# Autodesk Inventor assembly: DesignRootModel^PCB_ESP32-C3-MINI-1_V1(2)_PCB_ESP32-C3-MINI-1_V1
(part 2 of 3)
- C:\Users\micyg\Projects\virtual_pet\VirtualBlob\Mechanical\boards\MainBoard\MainBoard_0_4_0\VirtualBlob_MainBoard_0.4.0\VirtualBlob_MainBoard_0.4.0\uid__1-169^DesignRootModel_PCB_ESP32-C3-MINI-1_V1(2)_PCB_ESP32.ipt
- C:\Users\micyg\Projects\virtual_pet\VirtualBlob\Mechanical\boards\MainBoard\MainBoard_0_4_0\VirtualBlob_MainBoard_0.4.0\VirtualBlob_MainBoard_0.4.0\uid__1-170^DesignRootModel_PCB_ESP32-C3-MINI-1_V1(2)_PCB_ESP32.ipt
- C:\Users\micyg\Projects\virtual_pet\VirtualBlob\Mechanical\boards\MainBoard\MainBoard_0_4_0\VirtualBlob_MainBoard_0.4.0\VirtualBlob_MainBoard_0.4.0\uid__1-171^DesignRootModel_PCB_ESP32-C3-MINI-1_V1(2)_PCB_ESP32.ipt
- C:\Users\micyg\Projects\virtual_pet\VirtualBlob\Mechanical\boards\MainBoard\MainBoard_0_4_0\VirtualBlob_MainBoard_0.4.0\VirtualBlob_MainBoard_0.4.0\uid__1-172^DesignRootModel_PCB_ESP32-C3-MINI-1_V1(2)_PCB_ESP32.ipt
- C:\Users\micyg\Projects\virtual_pet\VirtualBlob\Mechanical\boards\MainBoard\MainBoard_0_4_0\VirtualBlob_MainBoard_0.4.0\VirtualBlob_MainBoard_0.4.0\uid__1-173^DesignRootModel_PCB_ESP32-C3-MINI-1_V1(2)_PCB_ESP32.ipt
- C:\Users\micyg\Projects\virtual_pet\VirtualBlob\Mechanical\boards\MainBoard\MainBoard_0_4_0\VirtualBlob_MainBoard_0.4.0\VirtualBlob_MainBoard_0.4.0\uid__1-174^DesignRootModel_PCB_ESP32-C3-MINI-1_V1(2)_PCB_ESP32.ipt
- C:\Users\micyg\Projects\virtual_pet\VirtualBlob\Mechanical\boards\MainBoard\MainBoard_0_4_0\VirtualBlob_MainBoard_0.4.0\VirtualBlob_MainBoard_0.4.0\uid__1-175^DesignRootModel_PCB_ESP32-C3-MINI-1_V1(2)_PCB_ESP32.ipt
- C:\Users\micyg\Projects\virtual_pet\VirtualBlob\Mechanical\boards\MainBoard\MainBoard_0_4_0\VirtualBlob_MainBoard_0.4.0\VirtualBlob_MainBoard_0.4.0\uid__1-176^DesignRootModel_PCB_ESP32-C3-MINI-1_V1(2)_PCB_ESP32.ipt
- C:\Users\micyg\Projects\virtual_pet\VirtualBlob\Mechanical\boards\MainBoard\MainBoard_0_4_0\VirtualBlob_MainBoard_0.4.0\VirtualBlob_MainBoard_0.4.0\uid__1-177^DesignRootModel_PCB_ESP32-C3-MINI-1_V1(2)_PCB_ESP32.ipt
- C:\Users\micyg\Projects\virtual_pet\VirtualBlob\Mechanical\boards\MainBoard\MainBoard_0_4_0\VirtualBlob_MainBoard_0.4.0\VirtualBlob_MainBoard_0.4.0\uid__1-178^DesignRootModel_PCB_ESP32-C3-MINI-1_V1(2)_PCB_ESP32.ipt
- C:\Users\micyg\Projects\virtual_pet\VirtualBlob\Mechanical\boards\MainBoard\MainBoard_0_4_0\VirtualBlob_MainBoard_0.4.0\VirtualBlob_MainBoard_0.4.0\uid__1-179^DesignRootModel_PCB_ESP32-C3-MINI-1_V1(2)_PCB_ESP32.ipt
- C:\Users\micyg\Projects\virtual_pet\VirtualBlob\Mechanical\boards\MainBoard\MainBoard_0_4_0\VirtualBlob_MainBoard_0.4.0\VirtualBlob_MainBoard_0.4.0\uid__1-180^DesignRootModel_PCB_ESP32-C3-MINI-1_V1(2)_PCB_ESP32.ipt
- C:\Users\micyg\Projects\virtual_pet\VirtualBlob\Mechanical\boards\MainBoard\MainBoard_0_4_0\VirtualBlob_MainBoard_0.4.0\VirtualBlob_MainBoard_0.4.0\uid__1-181^DesignRootModel_PCB_ESP32-C3-MINI-1_V1(2)_PCB_ESP32.ipt
- C:\Users\micyg\Projects\virtual_pet\VirtualBlob\Mechanical\boards\MainBoard\MainBoard_0_4_0\VirtualBlob_MainBoard_0.4.0\VirtualBlob_MainBoard_0.4.0\uid__1-182^DesignRootModel_PCB_ESP32-C3-MINI-1_V1(2)_PCB_ESP32.ipt
- C:\Users\micyg\Projects\virtual_pet\VirtualBlob\Mechanical\boards\MainBoard\MainBoard_0_4_0\VirtualBlob_MainBoard_0.4.0\VirtualBlob_MainBoard_0.4.0\uid__1-183^DesignRootModel_PCB_ESP32-C3-MINI-1_V1(2)_PCB_ESP32.ipt
- C:\Users\micyg\Projects\virtual_pet\VirtualBlob\Mechanical\boards\MainBoard\MainBoard_0_4_0\VirtualBlob_MainBoard_0.4.0\VirtualBlob_MainBoard_0.4.0\uid__1-184^DesignRootModel_PCB_ESP32-C3-MINI-1_V1(2)_PCB_ESP32.ipt
- C:\Users\micyg\Projects\virtual_pet\VirtualBlob\Mechanical\boards\MainBoard\MainBoard_0_4_0\VirtualBlob_MainBoard_0.4.0\VirtualBlob_MainBoard_0.4.0\uid__1-185^DesignRootModel_PCB_ESP32-C3-MINI-1_V1(2)_PCB_ESP32.ipt
- C:\Users\micyg\Projects\virtual_pet\VirtualBlob\Mechanical\boards\MainBoard\MainBoard_0_4_0\VirtualBlob_MainBoard_0.4.0\VirtualBlob_MainBoard_0.4.0\uid__1-186^DesignRootModel_PCB_ESP32-C3-MINI-1_V1(2)_PCB_ESP32.ipt
- C:\Users\micyg\Projects\virtual_pet\VirtualBlob\Mechanical\boards\MainBoard\MainBoard_0_4_0\VirtualBlob_MainBoard_0.4.0\VirtualBlob_MainBoard_0.4.0\uid__1-187^DesignRootModel_PCB_ESP32-C3-MINI-1_V1(2)_PCB_ESP32.ipt
- C:\Users\micyg\Projects\virtual_pet\VirtualBlob\Mechanical\boards\MainBoard\MainBoard_0_4_0\VirtualBlob_MainBoard_0.4.0\VirtualBlob_MainBoard_0.4.0\uid__1-188^DesignRootModel_PCB_ESP32-C3-MINI-1_V1(2)_PCB_ESP32.ipt
- C:\Users\micyg\Projects\virtual_pet\VirtualBlob\Mechanical\boards\MainBoard\MainBoard_0_4_0\VirtualBlob_MainBoard_0.4.0\VirtualBlob_MainBoard_0.4.0\uid__1-189^DesignRootModel_PCB_ESP32-C3-MINI-1_V1(2)_PCB_ESP32.ipt
- C:\Users\micyg\Projects\virtual_pet\VirtualBlob\Mechanical\boards\MainBoard\MainBoard_0_4_0\VirtualBlob_MainBoard_0.4.0\VirtualBlob_MainBoard_0.4.0\uid__1-190^DesignRootModel_PCB_ESP32-C3-MINI-1_V1(2)_PCB_ESP32.ipt
- C:\Users\micyg\Projects\virtual_pet\VirtualBlob\Mechanical\boards\MainBoard\MainBoard_0_4_0\VirtualBlob_MainBoard_0.4.0\VirtualBlob_MainBoard_0.4.0\uid__1-191^DesignRootModel_PCB_ESP32-C3-MINI-1_V1(2)_PCB_ESP32.ipt
- C:\Users\micyg\Projects\virtual_pet\VirtualBlob\Mechanical\boards\MainBoard\MainBoard_0_4_0\VirtualBlob_MainBoard_0.4.0\VirtualBlob_MainBoard_0.4.0\uid__1-192^DesignRootModel_PCB_ESP32-C3-MINI-1_V1(2)_PCB_ESP32.ipt
- C:\Users\micyg\Projects\virtual_pet\VirtualBlob\Mechanical\boards\MainBoard\MainBoard_0_4_0\VirtualBlob_MainBoard_0.4.0\VirtualBlob_MainBoard_0.4.0\uid__1-193^DesignRootModel_PCB_ESP32-C3-MINI-1_V1(2)_PCB_ESP32.ipt
- C:\Users\micyg\Projects\virtual_pet\VirtualBlob\Mechanical\boards\MainBoard\MainBoard_0_4_0\VirtualBlob_MainBoard_0.4.0\VirtualBlob_MainBoard_0.4.0\uid__1-194^DesignRootModel_PCB_ESP32-C3-MINI-1_V1(2)_PCB_ESP32.ipt
- C:\Users\micyg\Projects\virtual_pet\VirtualBlob\Mechanical\boards\MainBoard\MainBoard_0_4_0\VirtualBlob_MainBoard_0.4.0\VirtualBlob_MainBoard_0.4.0\uid__1-195^DesignRootModel_PCB_ESP32-C3-MINI-1_V1(2)_PCB_ESP32.ipt
- C:\Users\micyg\Projects\virtual_pet\VirtualBlob\Mechanical\boards\MainBoard\MainBoard_0_4_0\VirtualBlob_MainBoard_0.4.0\VirtualBlob_MainBoard_0.4.0\uid__1-196^DesignRootModel_PCB_ESP32-C3-MINI-1_V1(2)_PCB_ESP32.ipt
- C:\Users\micyg\Projects\virtual_pet\VirtualBlob\Mechanical\boards\MainBoard\MainBoard_0_4_0\VirtualBlob_MainBoard_0.4.0\VirtualBlob_MainBoard_0.4.0\uid__1-197^DesignRootModel_PCB_ESP32-C3-MINI-1_V1(2)_PCB_ESP32.ipt
- C:\Users\micyg\Projects\virtual_pet\VirtualBlob\Mechanical\boards\MainBoard\MainBoard_0_4_0\VirtualBlob_MainBoard_0.4.0\VirtualBlob_MainBoard_0.4.0\uid__1-198^DesignRootModel_PCB_ESP32-C3-MINI-1_V1(2)_PCB_ESP32.ipt
- C:\Users\micyg\Projects\virtual_pet\VirtualBlob\Mechanical\boards\MainBoard\MainBoard_0_4_0\VirtualBlob_MainBoard_0.4.0\VirtualBlob_MainBoard_0.4.0\uid__1-199^DesignRootModel_PCB_ESP32-C3-MINI-1_V1(2)_PCB_ESP32.ipt
- C:\Users\micyg\Projects\virtual_pet\VirtualBlob\Mechanical\boards\MainBoard\MainBoard_0_4_0\VirtualBlob_MainBoard_0.4.0\VirtualBlob_MainBoard_0.4.0\uid__1-200^DesignRootModel_PCB_ESP32-C3-MINI-1_V1(2)_PCB_ESP32.ipt
- C:\Users\micyg\Projects\virtual_pet\VirtualBlob\Mechanical\boards\MainBoard\MainBoard_0_4_0\VirtualBlob_MainBoard_0.4.0\VirtualBlob_MainBoard_0.4.0\uid__1-201^DesignRootModel_PCB_ESP32-C3-MINI-1_V1(2)_PCB_ESP32.ipt
- C:\Users\micyg\Projects\virtual_pet\VirtualBlob\Mechanical\boards\MainBoard\MainBoard_0_4_0\VirtualBlob_MainBoard_0.4.0\VirtualBlob_MainBoard_0.4.0\uid__1-202^DesignRootModel_PCB_ESP32-C3-MINI-1_V1(2)_PCB_ESP32.ipt
- C:\Users\micyg\Projects\virtual_pet\VirtualBlob\Mechanical\boards\MainBoard\MainBoard_0_4_0\VirtualBlob_MainBoard_0.4.0\VirtualBlob_MainBoard_0.4.0\uid__1-203^DesignRootModel_PCB_ESP32-C3-MINI-1_V1(2)_PCB_ESP32.ipt
- C:\Users\micyg\Projects\virtual_pet\VirtualBlob\Mechanical\boards\MainBoard\MainBoard_0_4_0\VirtualBlob_MainBoard_0.4.0\VirtualBlob_MainBoard_0.4.0\uid__1-204^DesignRootModel_PCB_ESP32-C3-MINI-1_V1(2)_PCB_ESP32.ipt
- C:\Users\micyg\Projects\virtual_pet\VirtualBlob\Mechanical\boards\MainBoard\MainBoard_0_4_0\VirtualBlob_MainBoard_0.4.0\VirtualBlob_MainBoard_0.4.0\uid__1-205^DesignRootModel_PCB_ESP32-C3-MINI-1_V1(2)_PCB_ESP32.ipt
- C:\Users\micyg\Projects\virtual_pet\VirtualBlob\Mechanical\boards\MainBoard\MainBoard_0_4_0\VirtualBlob_MainBoard_0.4.0\VirtualBlob_MainBoard_0.4.0\uid__1-206^DesignRootModel_PCB_ESP32-C3-MINI-1_V1(2)_PCB_ESP32.ipt
- C:\Users\micyg\Projects\virtual_pet\VirtualBlob\Mechanical\boards\MainBoard\MainBoard_0_4_0\VirtualBlob_MainBoard_0.4.0\VirtualBlob_MainBoard_0.4.0\uid__1-207^DesignRootModel_PCB_ESP32-C3-MINI-1_V1(2)_PCB_ESP32.ipt
- C:\Users\micyg\Projects\virtual_pet\VirtualBlob\Mechanical\boards\MainBoard\MainBoard_0_4_0\VirtualBlob_MainBoard_0.4.0\VirtualBlob_MainBoard_0.4.0\uid__1-208^DesignRootModel_PCB_ESP32-C3-MINI-1_V1(2)_PCB_ESP32.ipt
- C:\Users\micyg\Projects\virtual_pet\VirtualBlob\Mechanical\boards\MainBoard\MainBoard_0_4_0\VirtualBlob_MainBoard_0.4.0\VirtualBlob_MainBoard_0.4.0\uid__1-209^DesignRootModel_PCB_ESP32-C3-MINI-1_V1(2)_PCB_ESP32.ipt
- C:\Users\micyg\Projects\virtual_pet\VirtualBlob\Mechanical\boards\MainBoard\MainBoard_0_4_0\VirtualBlob_MainBoard_0.4.0\VirtualBlob_MainBoard_0.4.0\uid__1-210^DesignRootModel_PCB_ESP32-C3-MINI-1_V1(2)_PCB_ESP32.ipt
- C:\Users\micyg\Projects\virtual_pet\VirtualBlob\Mechanical\boards\MainBoard\MainBoard_0_4_0\VirtualBlob_MainBoard_0.4.0\VirtualBlob_MainBoard_0.4.0\uid__1-211^DesignRootModel_PCB_ESP32-C3-MINI-1_V1(2)_PCB_ESP32.ipt
- C:\Users\micyg\Projects\virtual_pet\VirtualBlob\Mechanical\boards\MainBoard\MainBoard_0_4_0\VirtualBlob_MainBoard_0.4.0\VirtualBlob_MainBoard_0.4.0\uid__1-212^DesignRootModel_PCB_ESP32-C3-MINI-1_V1(2)_PCB_ESP32.ipt
- C:\Users\micyg\Projects\virtual_pet\VirtualBlob\Mechanical\boards\MainBoard\MainBoard_0_4_0\VirtualBlob_MainBoard_0.4.0\VirtualBlob_MainBoard_0.4.0\uid__1-213^DesignRootModel_PCB_ESP32-C3-MINI-1_V1(2)_PCB_ESP32.ipt
- C:\Users\micyg\Projects\virtual_pet\VirtualBlob\Mechanical\boards\MainBoard\MainBoard_0_4_0\VirtualBlob_MainBoard_0.4.0\VirtualBlob_MainBoard_0.4.0\uid__1-214^DesignRootModel_PCB_ESP32-C3-MINI-1_V1(2)_PCB_ESP32.ipt
- C:\Users\micyg\Projects\virtual_pet\VirtualBlob\Mechanical\boards\MainBoard\MainBoard_0_4_0\VirtualBlob_MainBoard_0.4.0\VirtualBlob_MainBoard_0.4.0\uid__1-215^DesignRootModel_PCB_ESP32-C3-MINI-1_V1(2)_PCB_ESP32.ipt
- C:\Users\micyg\Projects\virtual_pet\VirtualBlob\Mechanical\boards\MainBoard\MainBoard_0_4_0\VirtualBlob_MainBoard_0.4.0\VirtualBlob_MainBoard_0.4.0\uid__1-216^DesignRootModel_PCB_ESP32-C3-MINI-1_V1(2)_PCB_ESP32.ipt
- C:\Users\micyg\Projects\virtual_pet\VirtualBlob\Mechanical\boards\MainBoard\MainBoard_0_4_0\VirtualBlob_MainBoard_0.4.0\VirtualBlob_MainBoard_0.4.0\uid__1-217^DesignRootModel_PCB_ESP32-C3-MINI-1_V1(2)_PCB_ESP32.ipt
- C:\Users\micyg\Projects\virtual_pet\VirtualBlob\Mechanical\boards\MainBoard\MainBoard_0_4_0\VirtualBlob_MainBoard_0.4.0\VirtualBlob_MainBoard_0.4.0\uid__1-218^DesignRootModel_PCB_ESP32-C3-MINI-1_V1(2)_PCB_ESP32.ipt
- C:\Users\micyg\Projects\virtual_pet\VirtualBlob\Mechanical\boards\MainBoard\MainBoard_0_4_0\VirtualBlob_MainBoard_0.4.0\VirtualBlob_MainBoard_0.4.0\uid__1-219^DesignRootModel_PCB_ESP32-C3-MINI-1_V1(2)_PCB_ESP32.ipt
- C:\Users\micyg\Projects\virtual_pet\VirtualBlob\Mechanical\boards\MainBoard\MainBoard_0_4_0\VirtualBlob_MainBoard_0.4.0\VirtualBlob_MainBoard_0.4.0\uid__1-220^DesignRootModel_PCB_ESP32-C3-MINI-1_V1(2)_PCB_ESP32.ipt
- C:\Users\micyg\Projects\virtual_pet\VirtualBlob\Mechanical\boards\MainBoard\MainBoard_0_4_0\VirtualBlob_MainBoard_0.4.0\VirtualBlob_MainBoard_0.4.0\uid__1-221^DesignRootModel_PCB_ESP32-C3-MINI-1_V1(2)_PCB_ESP32.ipt
- C:\Users\micyg\Projects\virtual_pet\VirtualBlob\Mechanical\boards\MainBoard\MainBoard_0_4_0\VirtualBlob_MainBoard_0.4.0\VirtualBlob_MainBoard_0.4.0\uid__1-222^DesignRootModel_PCB_ESP32-C3-MINI-1_V1(2)_PCB_ESP32.ipt
- C:\Users\micyg\Projects\virtual_pet\VirtualBlob\Mechanical\boards\MainBoard\MainBoard_0_4_0\VirtualBlob_MainBoard_0.4.0\VirtualBlob_MainBoard_0.4.0\uid__1-223^DesignRootModel_PCB_ESP32-C3-MINI-1_V1(2)_PCB_ESP32.ipt
- C:\Users\micyg\Projects\virtual_pet\VirtualBlob\Mechanical\boards\MainBoard\MainBoard_0_4_0\VirtualBlob_MainBoard_0.4.0\VirtualBlob_MainBoard_0.4.0\uid__1-224^DesignRootModel_PCB_ESP32-C3-MINI-1_V1(2)_PCB_ESP32.ipt
- C:\Users\micyg\Projects\virtual_pet\VirtualBlob\Mechanical\boards\MainBoard\MainBoard_0_4_0\VirtualBlob_MainBoard_0.4.0\VirtualBlob_MainBoard_0.4.0\uid__1-225^DesignRootModel_PCB_ESP32-C3-MINI-1_V1(2)_PCB_ESP32.ipt
- C:\Users\micyg\Projects\virtual_pet\VirtualBlob\Mechanical\boards\MainBoard\MainBoard_0_4_0\VirtualBlob_MainBoard_0.4.0\VirtualBlob_MainBoard_0.4.0\uid__1-226^DesignRootModel_PCB_ESP32-C3-MINI-1_V1(2)_PCB_ESP32.ipt
- C:\Users\micyg\Projects\virtual_pet\VirtualBlob\Mechanical\boards\MainBoard\MainBoard_0_4_0\VirtualBlob_MainBoard_0.4.0\VirtualBlob_MainBoard_0.4.0\uid__1-227^DesignRootModel_PCB_ESP32-C3-MINI-1_V1(2)_PCB_ESP32.ipt
- C:\Users\micyg\Projects\virtual_pet\VirtualBlob\Mechanical\boards\MainBoard\MainBoard_0_4_0\VirtualBlob_MainBoard_0.4.0\VirtualBlob_MainBoard_0.4.0\uid__1-228^DesignRootModel_PCB_ESP32-C3-MINI-1_V1(2)_PCB_ESP32.ipt
- C:\Users\micyg\Projects\virtual_pet\VirtualBlob\Mechanical\boards\MainBoard\MainBoard_0_4_0\VirtualBlob_MainBoard_0.4.0\VirtualBlob_MainBoard_0.4.0\uid__1-229^DesignRootModel_PCB_ESP32-C3-MINI-1_V1(2)_PCB_ESP32.ipt
- C:\Users\micyg\Projects\virtual_pet\VirtualBlob\Mechanical\boards\MainBoard\MainBoard_0_4_0\VirtualBlob_MainBoard_0.4.0\VirtualBlob_MainBoard_0.4.0\uid__1-230^DesignRootModel_PCB_ESP32-C3-MINI-1_V1(2)_PCB_ESP32.ipt
- C:\Users\micyg\Projects\virtual_pet\VirtualBlob\Mechanical\boards\MainBoard\MainBoard_0_4_0\VirtualBlob_MainBoard_0.4.0\VirtualBlob_MainBoard_0.4.0\uid__1-231^DesignRootModel_PCB_ESP32-C3-MINI-1_V1(2)_PCB_ESP32.ipt
- C:\Users\micyg\Projects\virtual_pet\VirtualBlob\Mechanical\boards\MainBoard\MainBoard_0_4_0\VirtualBlob_MainBoard_0.4.0\VirtualBlob_MainBoard_0.4.0\uid__1-232^DesignRootModel_PCB_ESP32-C3-MINI-1_V1(2)_PCB_ESP32.ipt
- C:\Users\micyg\Projects\virtual_pet\VirtualBlob\Mechanical\boards\MainBoard\MainBoard_0_4_0\VirtualBlob_MainBoard_0.4.0\VirtualBlob_MainBoard_0.4.0\uid__1-233^DesignRootModel_PCB_ESP32-C3-MINI-1_V1(2)_PCB_ESP32.ipt
- C:\Users\micyg\Projects\virtual_pet\VirtualBlob\Mechanical\boards\MainBoard\MainBoard_0_4_0\VirtualBlob_MainBoard_0.4.0\VirtualBlob_MainBoard_0.4.0\uid__1-234^DesignRootModel_PCB_ESP32-C3-MINI-1_V1(2)_PCB_ESP32.ipt
- C:\Users\micyg\Projects\virtual_pet\VirtualBlob\Mechanical\boards\MainBoard\MainBoard_0_4_0\VirtualBlob_MainBoard_0.4.0\VirtualBlob_MainBoard_0.4.0\uid__1-235^DesignRootModel_PCB_ESP32-C3-MINI-1_V1(2)_PCB_ESP32.ipt
- C:\Users\micyg\Projects\virtual_pet\VirtualBlob\Mechanical\boards\MainBoard\MainBoard_0_4_0\VirtualBlob_MainBoard_0.4.0\VirtualBlob_MainBoard_0.4.0\uid__1-236^DesignRootModel_PCB_ESP32-C3-MINI-1_V1(2)_PCB_ESP32.ipt
- C:\Users\micyg\Projects\virtual_pet\VirtualBlob\Mechanical\boards\MainBoard\MainBoard_0_4_0\VirtualBlob_MainBoard_0.4.0\VirtualBlob_MainBoard_0.4.0\uid__1-237^DesignRootModel_PCB_ESP32-C3-MINI-1_V1(2)_PCB_ESP32.ipt
- C:\Users\micyg\Projects\virtual_pet\VirtualBlob\Mechanical\boards\MainBoard\MainBoard_0_4_0\VirtualBlob_MainBoard_0.4.0\VirtualBlob_MainBoard_0.4.0\uid__1-238^DesignRootModel_PCB_ESP32-C3-MINI-1_V1(2)_PCB_ESP32.ipt
- C:\Users\micyg\Projects\virtual_pet\VirtualBlob\Mechanical\boards\MainBoard\MainBoard_0_4_0\VirtualBlob_MainBoard_0.4.0\VirtualBlob_MainBoard_0.4.0\uid__1-239^DesignRootModel_PCB_ESP32-C3-MINI-1_V1(2)_PCB_ESP32.ipt
- C:\Users\micyg\Projects\virtual_pet\VirtualBlob\Mechanical\boards\MainBoard\MainBoard_0_4_0\VirtualBlob_MainBoard_0.4.0\VirtualBlob_MainBoard_0.4.0\uid__1-240^DesignRootModel_PCB_ESP32-C3-MINI-1_V1(2)_PCB_ESP32.ipt
- C:\Users\micyg\Projects\virtual_pet\VirtualBlob\Mechanical\boards\MainBoard\MainBoard_0_4_0\VirtualBlob_MainBoard_0.4.0\VirtualBlob_MainBoard_0.4.0\uid__1-241^DesignRootModel_PCB_ESP32-C3-MINI-1_V1(2)_PCB_ESP32.ipt
- C:\Users\micyg\Projects\virtual_pet\VirtualBlob\Mechanical\boards\MainBoard\MainBoard_0_4_0\VirtualBlob_MainBoard_0.4.0\VirtualBlob_MainBoard_0.4.0\uid__1-242^DesignRootModel_PCB_ESP32-C3-MINI-1_V1(2)_PCB_ESP32.ipt
- C:\Users\micyg\Projects\virtual_pet\VirtualBlob\Mechanical\boards\MainBoard\MainBoard_0_4_0\VirtualBlob_MainBoard_0.4.0\VirtualBlob_MainBoard_0.4.0\uid__1-243^DesignRootModel_PCB_ESP32-C3-MINI-1_V1(2)_PCB_ESP32.ipt
- C:\Users\micyg\Projects\virtual_pet\VirtualBlob\Mechanical\boards\MainBoard\MainBoard_0_4_0\VirtualBlob_MainBoard_0.4.0\VirtualBlob_MainBoard_0.4.0\uid__1-244^DesignRootModel_PCB_ESP32-C3-MINI-1_V1(2)_PCB_ESP32.ipt
- C:\Users\micyg\Projects\virtual_pet\VirtualBlob\Mechanical\boards\MainBoard\MainBoard_0_4_0\VirtualBlob_MainBoard_0.4.0\VirtualBlob_MainBoard_0.4.0\uid__1-245^DesignRootModel_PCB_ESP32-C3-MINI-1_V1(2)_PCB_ESP32.ipt
- C:\Users\micyg\Projects\virtual_pet\VirtualBlob\Mechanical\boards\MainBoard\MainBoard_0_4_0\VirtualBlob_MainBoard_0.4.0\VirtualBlob_MainBoard_0.4.0\uid__1-246^DesignRootModel_PCB_ESP32-C3-MINI-1_V1(2)_PCB_ESP32.ipt
- C:\Users\micyg\Projects\virtual_pet\VirtualBlob\Mechanical\boards\MainBoard\MainBoard_0_4_0\VirtualBlob_MainBoard_0.4.0\VirtualBlob_MainBoard_0.4.0\uid__1-247^DesignRootModel_PCB_ESP32-C3-MINI-1_V1(2)_PCB_ESP32.ipt
- C:\Users\micyg\Projects\virtual_pet\VirtualBlob\Mechanical\boards\MainBoard\MainBoard_0_4_0\VirtualBlob_MainBoard_0.4.0\VirtualBlob_MainBoard_0.4.0\uid__1-248^DesignRootModel_PCB_ESP32-C3-MINI-1_V1(2)_PCB_ESP32.ipt
- C:\Users\micyg\Projects\virtual_pet\VirtualBlob\Mechanical\boards\MainBoard\MainBoard_0_4_0\VirtualBlob_MainBoard_0.4.0\VirtualBlob_MainBoard_0.4.0\uid__1-249^DesignRootModel_PCB_ESP32-C3-MINI-1_V1(2)_PCB_ESP32.ipt
- C:\Users\micyg\Projects\virtual_pet\VirtualBlob\Mechanical\boards\MainBoard\MainBoard_0_4_0\VirtualBlob_MainBoard_0.4.0\VirtualBlob_MainBoard_0.4.0\uid__1-250^DesignRootModel_PCB_ESP32-C3-MINI-1_V1(2)_PCB_ESP32.ipt
- C:\Users\micyg\Projects\virtual_pet\VirtualBlob\Mechanical\boards\MainBoard\MainBoard_0_4_0\VirtualBlob_MainBoard_0.4.0\VirtualBlob_MainBoard_0.4.0\uid__1-251^DesignRootModel_PCB_ESP32-C3-MINI-1_V1(2)_PCB_ESP32.ipt
- C:\Users\micyg\Projects\virtual_pet\VirtualBlob\Mechanical\boards\MainBoard\MainBoard_0_4_0\VirtualBlob_MainBoard_0.4.0\VirtualBlob_MainBoard_0.4.0\uid__1-252^DesignRootModel_PCB_ESP32-C3-MINI-1_V1(2)_PCB_ESP32.ipt
- C:\Users\micyg\Projects\virtual_pet\VirtualBlob\Mechanical\boards\MainBoard\MainBoard_0_4_0\VirtualBlob_MainBoard_0.4.0\VirtualBlob_MainBoard_0.4.0\uid__1-253^DesignRootModel_PCB_ESP32-C3-MINI-1_V1(2)_PCB_ESP32.ipt
- C:\Users\micyg\Projects\virtual_pet\VirtualBlob\Mechanical\boards\MainBoard\MainBoard_0_4_0\VirtualBlob_MainBoard_0.4.0\VirtualBlob_MainBoard_0.4.0\uid__1-254^DesignRootModel_PCB_ESP32-C3-MINI-1_V1(2)_PCB_ESP32.ipt
- C:\Users\micyg\Projects\virtual_pet\VirtualBlob\Mechanical\boards\MainBoard\MainBoard_0_4_0\VirtualBlob_MainBoard_0.4.0\VirtualBlob_MainBoard_0.4.0\uid__1-255^DesignRootModel_PCB_ESP32-C3-MINI-1_V1(2)_PCB_ESP32.ipt
- C:\Users\micyg\Projects\virtual_pet\VirtualBlob\Mechanical\boards\MainBoard\MainBoard_0_4_0\VirtualBlob_MainBoard_0.4.0\VirtualBlob_MainBoard_0.4.0\uid__1-256^DesignRootModel_PCB_ESP32-C3-MINI-1_V1(2)_PCB_ESP32.ipt
- C:\Users\micyg\Projects\virtual_pet\VirtualBlob\Mechanical\boards\MainBoard\MainBoard_0_4_0\VirtualBlob_MainBoard_0.4.0\VirtualBlob_MainBoard_0.4.0\uid__1-257^DesignRootModel_PCB_ESP32-C3-MINI-1_V1(2)_PCB_ESP32.ipt
- C:\Users\micyg\Projects\virtual_pet\VirtualBlob\Mechanical\boards\MainBoard\MainBoard_0_4_0\VirtualBlob_MainBoard_0.4.0\VirtualBlob_MainBoard_0.4.0\uid__1-258^DesignRootModel_PCB_ESP32-C3-MINI-1_V1(2)_PCB_ESP32.ipt
- C:\Users\micyg\Projects\virtual_pet\VirtualBlob\Mechanical\boards\MainBoard\MainBoard_0_4_0\VirtualBlob_MainBoard_0.4.0\VirtualBlob_MainBoard_0.4.0\uid__1-259^DesignRootModel_PCB_ESP32-C3-MINI-1_V1(2)_PCB_ESP32.ipt
- C:\Users\micyg\Projects\virtual_pet\VirtualBlob\Mechanical\boards\MainBoard\MainBoard_0_4_0\VirtualBlob_MainBoard_0.4.0\VirtualBlob_MainBoard_0.4.0\uid__1-260^DesignRootModel_PCB_ESP32-C3-MINI-1_V1(2)_PCB_ESP32.ipt
- C:\Users\micyg\Projects\virtual_pet\VirtualBlob\Mechanical\boards\MainBoard\MainBoard_0_4_0\VirtualBlob_MainBoard_0.4.0\VirtualBlob_MainBoard_0.4.0\uid__1-261^DesignRootModel_PCB_ESP32-C3-MINI-1_V1(2)_PCB_ESP32.ipt
- C:\Users\micyg\Projects\virtual_pet\VirtualBlob\Mechanical\boards\MainBoard\MainBoard_0_4_0\VirtualBlob_MainBoard_0.4.0\VirtualBlob_MainBoard_0.4.0\uid__1-262^DesignRootModel_PCB_ESP32-C3-MINI-1_V1(2)_PCB_ESP32.ipt
- C:\Users\micyg\Projects\virtual_pet\VirtualBlob\Mechanical\boards\MainBoard\MainBoard_0_4_0\VirtualBlob_MainBoard_0.4.0\VirtualBlob_MainBoard_0.4.0\uid__1-263^DesignRootModel_PCB_ESP32-C3-MINI-1_V1(2)_PCB_ESP32.ipt
- C:\Users\micyg\Projects\virtual_pet\VirtualBlob\Mechanical\boards\MainBoard\MainBoard_0_4_0\VirtualBlob_MainBoard_0.4.0\VirtualBlob_MainBoard_0.4.0\uid__1-264^DesignRootModel_PCB_ESP32-C3-MINI-1_V1(2)_PCB_ESP32.ipt
- C:\Users\micyg\Projects\virtual_pet\VirtualBlob\Mechanical\boards\MainBoard\MainBoard_0_4_0\VirtualBlob_MainBoard_0.4.0\VirtualBlob_MainBoard_0.4.0\uid__1-265^DesignRootModel_PCB_ESP32-C3-MINI-1_V1(2)_PCB_ESP32.ipt
- C:\Users\micyg\Projects\virtual_pet\VirtualBlob\Mechanical\boards\MainBoard\MainBoard_0_4_0\VirtualBlob_MainBoard_0.4.0\VirtualBlob_MainBoard_0.4.0\uid__1-266^DesignRootModel_PCB_ESP32-C3-MINI-1_V1(2)_PCB_ESP32.ipt
- C:\Users\micyg\Projects\virtual_pet\VirtualBlob\Mechanical\boards\MainBoard\MainBoard_0_4_0\VirtualBlob_MainBoard_0.4.0\VirtualBlob_MainBoard_0.4.0\uid__1-267^DesignRootModel_PCB_ESP32-C3-MINI-1_V1(2)_PCB_ESP32.ipt
- C:\Users\micyg\Projects\virtual_pet\VirtualBlob\Mechanical\boards\MainBoard\MainBoard_0_4_0\VirtualBlob_MainBoard_0.4.0\VirtualBlob_MainBoard_0.4.0\uid__1-268^DesignRootModel_PCB_ESP32-C3-MINI-1_V1(2)_PCB_ESP32.ipt
- C:\Users\micyg\Projects\virtual_pet\VirtualBlob\Mechanical\boards\MainBoard\MainBoard_0_4_0\VirtualBlob_MainBoard_0.4.0\VirtualBlob_MainBoard_0.4.0\uid__1-269^DesignRootModel_PCB_ESP32-C3-MINI-1_V1(2)_PCB_ESP32.ipt
- C:\Users\micyg\Projects\virtual_pet\VirtualBlob\Mechanical\boards\MainBoard\MainBoard_0_4_0\VirtualBlob_MainBoard_0.4.0\VirtualBlob_MainBoard_0.4.0\uid__1-270^DesignRootModel_PCB_ESP32-C3-MINI-1_V1(2)_PCB_ESP32.ipt
- C:\Users\micyg\Projects\virtual_pet\VirtualBlob\Mechanical\boards\MainBoard\MainBoard_0_4_0\VirtualBlob_MainBoard_0.4.0\VirtualBlob_MainBoard_0.4.0\uid__1-271^DesignRootModel_PCB_ESP32-C3-MINI-1_V1(2)_PCB_ESP32.ipt
- C:\Users\micyg\Projects\virtual_pet\VirtualBlob\Mechanical\boards\MainBoard\MainBoard_0_4_0\VirtualBlob_MainBoard_0.4.0\VirtualBlob_MainBoard_0.4.0\uid__1-272^DesignRootModel_PCB_ESP32-C3-MINI-1_V1(2)_PCB_ESP32.ipt
- C:\Users\micyg\Projects\virtual_pet\VirtualBlob\Mechanical\boards\MainBoard\MainBoard_0_4_0\VirtualBlob_MainBoard_0.4.0\VirtualBlob_MainBoard_0.4.0\uid__1-273^DesignRootModel_PCB_ESP32-C3-MINI-1_V1(2)_PCB_ESP32.ipt
- C:\Users\micyg\Projects\virtual_pet\VirtualBlob\Mechanical\boards\MainBoard\MainBoard_0_4_0\VirtualBlob_MainBoard_0.4.0\VirtualBlob_MainBoard_0.4.0\uid__1-274^DesignRootModel_PCB_ESP32-C3-MINI-1_V1(2)_PCB_ESP32.ipt
- C:\Users\micyg\Projects\virtual_pet\VirtualBlob\Mechanical\boards\MainBoard\MainBoard_0_4_0\VirtualBlob_MainBoard_0.4.0\VirtualBlob_MainBoard_0.4.0\uid__1-275^DesignRootModel_PCB_ESP32-C3-MINI-1_V1(2)_PCB_ESP32.ipt
- C:\Users\micyg\Projects\virtual_pet\VirtualBlob\Mechanical\boards\MainBoard\MainBoard_0_4_0\VirtualBlob_MainBoard_0.4.0\VirtualBlob_MainBoard_0.4.0\uid__1-276^DesignRootModel_PCB_ESP32-C3-MINI-1_V1(2)_PCB_ESP32.ipt
- C:\Users\micyg\Projects\virtual_pet\VirtualBlob\Mechanical\boards\MainBoard\MainBoard_0_4_0\VirtualBlob_MainBoard_0.4.0\VirtualBlob_MainBoard_0.4.0\uid__1-277^DesignRootModel_PCB_ESP32-C3-MINI-1_V1(2)_PCB_ESP32.ipt
- C:\Users\micyg\Projects\virtual_pet\VirtualBlob\Mechanical\boards\MainBoard\MainBoard_0_4_0\VirtualBlob_MainBoard_0.4.0\VirtualBlob_MainBoard_0.4.0\uid__1-278^DesignRootModel_PCB_ESP32-C3-MINI-1_V1(2)_PCB_ESP32.ipt
- C:\Users\micyg\Projects\virtual_pet\VirtualBlob\Mechanical\boards\MainBoard\MainBoard_0_4_0\VirtualBlob_MainBoard_0.4.0\VirtualBlob_MainBoard_0.4.0\uid__1-279^DesignRootModel_PCB_ESP32-C3-MINI-1_V1(2)_PCB_ESP32.ipt
- C:\Users\micyg\Projects\virtual_pet\VirtualBlob\Mechanical\boards\MainBoard\MainBoard_0_4_0\VirtualBlob_MainBoard_0.4.0\VirtualBlob_MainBoard_0.4.0\uid__1-280^DesignRootModel_PCB_ESP32-C3-MINI-1_V1(2)_PCB_ESP32.ipt
- C:\Users\micyg\Projects\virtual_pet\VirtualBlob\Mechanical\boards\MainBoard\MainBoard_0_4_0\VirtualBlob_MainBoard_0.4.0\VirtualBlob_MainBoard_0.4.0\uid__1-281^DesignRootModel_PCB_ESP32-C3-MINI-1_V1(2)_PCB_ESP32.ipt
- C:\Users\micyg\Projects\virtual_pet\VirtualBlob\Mechanical\boards\MainBoard\MainBoard_0_4_0\VirtualBlob_MainBoard_0.4.0\VirtualBlob_MainBoard_0.4.0\uid__1-282^DesignRootModel_PCB_ESP32-C3-MINI-1_V1(2)_PCB_ESP32.ipt
- C:\Users\micyg\Projects\virtual_pet\VirtualBlob\Mechanical\boards\MainBoard\MainBoard_0_4_0\VirtualBlob_MainBoard_0.4.0\VirtualBlob_MainBoard_0.4.0\uid__1-283^DesignRootModel_PCB_ESP32-C3-MINI-1_V1(2)_PCB_ESP32.ipt
- C:\Users\micyg\Projects\virtual_pet\VirtualBlob\Mechanical\boards\MainBoard\MainBoard_0_4_0\VirtualBlob_MainBoard_0.4.0\VirtualBlob_MainBoard_0.4.0\uid__1-284^DesignRootModel_PCB_ESP32-C3-MINI-1_V1(2)_PCB_ESP32.ipt
- C:\Users\micyg\Projects\virtual_pet\VirtualBlob\Mechanical\boards\MainBoard\MainBoard_0_4_0\VirtualBlob_MainBoard_0.4.0\VirtualBlob_MainBoard_0.4.0\uid__1-285^DesignRootModel_PCB_ESP32-C3-MINI-1_V1(2)_PCB_ESP32.ipt
- C:\Users\micyg\Projects\virtual_pet\VirtualBlob\Mechanical\boards\MainBoard\MainBoard_0_4_0\VirtualBlob_MainBoard_0.4.0\VirtualBlob_MainBoard_0.4.0\uid__1-286^DesignRootModel_PCB_ESP32-C3-MINI-1_V1(2)_PCB_ESP32.ipt
- C:\Users\micyg\Projects\virtual_pet\VirtualBlob\Mechanical\boards\MainBoard\MainBoard_0_4_0\VirtualBlob_MainBoard_0.4.0\VirtualBlob_MainBoard_0.4.0\uid__1-287^DesignRootModel_PCB_ESP32-C3-MINI-1_V1(2)_PCB_ESP32.ipt
- C:\Users\micyg\Projects\virtual_pet\VirtualBlob\Mechanical\boards\MainBoard\MainBoard_0_4_0\VirtualBlob_MainBoard_0.4.0\VirtualBlob_MainBoard_0.4.0\uid__1-288^DesignRootModel_PCB_ESP32-C3-MINI-1_V1(2)_PCB_ESP32.ipt
- C:\Users\micyg\Projects\virtual_pet\VirtualBlob\Mechanical\boards\MainBoard\MainBoard_0_4_0\VirtualBlob_MainBoard_0.4.0\VirtualBlob_MainBoard_0.4.0\uid__1-289^DesignRootModel_PCB_ESP32-C3-MINI-1_V1(2)_PCB_ESP32.ipt
- C:\Users\micyg\Projects\virtual_pet\VirtualBlob\Mechanical\boards\MainBoard\MainBoard_0_4_0\VirtualBlob_MainBoard_0.4.0\VirtualBlob_MainBoard_0.4.0\uid__1-290^DesignRootModel_PCB_ESP32-C3-MINI-1_V1(2)_PCB_ESP32.ipt
- C:\Users\micyg\Projects\virtual_pet\VirtualBlob\Mechanical\boards\MainBoard\MainBoard_0_4_0\VirtualBlob_MainBoard_0.4.0\VirtualBlob_MainBoard_0.4.0\uid__1-291^DesignRootModel_PCB_ESP32-C3-MINI-1_V1(2)_PCB_ESP32.ipt
- C:\Users\micyg\Projects\virtual_pet\VirtualBlob\Mechanical\boards\MainBoard\MainBoard_0_4_0\VirtualBlob_MainBoard_0.4.0\VirtualBlob_MainBoard_0.4.0\uid__1-292^DesignRootModel_PCB_ESP32-C3-MINI-1_V1(2)_PCB_ESP32.ipt
- C:\Users\micyg\Projects\virtual_pet\VirtualBlob\Mechanical\boards\MainBoard\MainBoard_0_4_0\VirtualBlob_MainBoard_0.4.0\VirtualBlob_MainBoard_0.4.0\uid__1-293^DesignRootModel_PCB_ESP32-C3-MINI-1_V1(2)_PCB_ESP32.ipt
- C:\Users\micyg\Projects\virtual_pet\VirtualBlob\Mechanical\boards\MainBoard\MainBoard_0_4_0\VirtualBlob_MainBoard_0.4.0\VirtualBlob_MainBoard_0.4.0\uid__1-294^DesignRootModel_PCB_ESP32-C3-MINI-1_V1(2)_PCB_ESP32.ipt
- C:\Users\micyg\Projects\virtual_pet\VirtualBlob\Mechanical\boards\MainBoard\MainBoard_0_4_0\VirtualBlob_MainBoard_0.4.0\VirtualBlob_MainBoard_0.4.0\uid__1-295^DesignRootModel_PCB_ESP32-C3-MINI-1_V1(2)_PCB_ESP32.ipt
- C:\Users\micyg\Projects\virtual_pet\VirtualBlob\Mechanical\boards\MainBoard\MainBoard_0_4_0\VirtualBlob_MainBoard_0.4.0\VirtualBlob_MainBoard_0.4.0\uid__1-296^DesignRootModel_PCB_ESP32-C3-MINI-1_V1(2)_PCB_ESP32.ipt
- C:\Users\micyg\Projects\virtual_pet\VirtualBlob\Mechanical\boards\MainBoard\MainBoard_0_4_0\VirtualBlob_MainBoard_0.4.0\VirtualBlob_MainBoard_0.4.0\uid__1-297^DesignRootModel_PCB_ESP32-C3-MINI-1_V1(2)_PCB_ESP32.ipt
- C:\Users\micyg\Projects\virtual_pet\VirtualBlob\Mechanical\boards\MainBoard\MainBoard_0_4_0\VirtualBlob_MainBoard_0.4.0\VirtualBlob_MainBoard_0.4.0\uid__1-298^DesignRootModel_PCB_ESP32-C3-MINI-1_V1(2)_PCB_ESP32.ipt
- C:\Users\micyg\Projects\virtual_pet\VirtualBlob\Mechanical\boards\MainBoard\MainBoard_0_4_0\VirtualBlob_MainBoard_0.4.0\VirtualBlob_MainBoard_0.4.0\uid__1-299^DesignRootModel_PCB_ESP32-C3-MINI-1_V1(2)_PCB_ESP32.ipt
- C:\Users\micyg\Projects\virtual_pet\VirtualBlob\Mechanical\boards\MainBoard\MainBoard_0_4_0\VirtualBlob_MainBoard_0.4.0\VirtualBlob_MainBoard_0.4.0\uid__1-300^DesignRootModel_PCB_ESP32-C3-MINI-1_V1(2)_PCB_ESP32.ipt
- C:\Users\micyg\Projects\virtual_pet\VirtualBlob\Mechanical\boards\MainBoard\MainBoard_0_4_0\VirtualBlob_MainBoard_0.4.0\VirtualBlob_MainBoard_0.4.0\uid__1-301^DesignRootModel_PCB_ESP32-C3-MINI-1_V1(2)_PCB_ESP32.ipt
- C:\Users\micyg\Projects\virtual_pet\VirtualBlob\Mechanical\boards\MainBoard\MainBoard_0_4_0\VirtualBlob_MainBoard_0.4.0\VirtualBlob_MainBoard_0.4.0\uid__1-302^DesignRootModel_PCB_ESP32-C3-MINI-1_V1(2)_PCB_ESP32.ipt
- C:\Users\micyg\Projects\virtual_pet\VirtualBlob\Mechanical\boards\MainBoard\MainBoard_0_4_0\VirtualBlob_MainBoard_0.4.0\VirtualBlob_MainBoard_0.4.0\uid__1-303^DesignRootModel_PCB_ESP32-C3-MINI-1_V1(2)_PCB_ESP32.ipt
- C:\Users\micyg\Projects\virtual_pet\VirtualBlob\Mechanical\boards\MainBoard\MainBoard_0_4_0\VirtualBlob_MainBoard_0.4.0\VirtualBlob_MainBoard_0.4.0\uid__1-304^DesignRootModel_PCB_ESP32-C3-MINI-1_V1(2)_PCB_ESP32.ipt
- C:\Users\micyg\Projects\virtual_pet\VirtualBlob\Mechanical\boards\MainBoard\MainBoard_0_4_0\VirtualBlob_MainBoard_0.4.0\VirtualBlob_MainBoard_0.4.0\uid__1-305^DesignRootModel_PCB_ESP32-C3-MINI-1_V1(2)_PCB_ESP32.ipt
- C:\Users\micyg\Projects\virtual_pet\VirtualBlob\Mechanical\boards\MainBoard\MainBoard_0_4_0\VirtualBlob_MainBoard_0.4.0\VirtualBlob_MainBoard_0.4.0\uid__1-306^DesignRootModel_PCB_ESP32-C3-MINI-1_V1(2)_PCB_ESP32.ipt
- C:\Users\micyg\Projects\virtual_pet\VirtualBlob\Mechanical\boards\MainBoard\MainBoard_0_4_0\VirtualBlob_MainBoard_0.4.0\VirtualBlob_MainBoard_0.4.0\uid__1-307^DesignRootModel_PCB_ESP32-C3-MINI-1_V1(2)_PCB_ESP32.ipt
- C:\Users\micyg\Projects\virtual_pet\VirtualBlob\Mechanical\boards\MainBoard\MainBoard_0_4_0\VirtualBlob_MainBoard_0.4.0\VirtualBlob_MainBoard_0.4.0\uid__1-308^DesignRootModel_PCB_ESP32-C3-MINI-1_V1(2)_PCB_ESP32.ipt
- C:\Users\micyg\Projects\virtual_pet\VirtualBlob\Mechanical\boards\MainBoard\MainBoard_0_4_0\VirtualBlob_MainBoard_0.4.0\VirtualBlob_MainBoard_0.4.0\uid__1-309^DesignRootModel_PCB_ESP32-C3-MINI-1_V1(2)_PCB_ESP32.ipt
- C:\Users\micyg\Projects\virtual_pet\VirtualBlob\Mechanical\boards\MainBoard\MainBoard_0_4_0\VirtualBlob_MainBoard_0.4.0\VirtualBlob_MainBoard_0.4.0\uid__1-310^DesignRootModel_PCB_ESP32-C3-MINI-1_V1(2)_PCB_ESP32.ipt
- C:\Users\micyg\Projects\virtual_pet\VirtualBlob\Mechanical\boards\MainBoard\MainBoard_0_4_0\VirtualBlob_MainBoard_0.4.0\VirtualBlob_MainBoard_0.4.0\uid__1-311^DesignRootModel_PCB_ESP32-C3-MINI-1_V1(2)_PCB_ESP32.ipt
- C:\Users\micyg\Projects\virtual_pet\VirtualBlob\Mechanical\boards\MainBoard\MainBoard_0_4_0\VirtualBlob_MainBoard_0.4.0\VirtualBlob_MainBoard_0.4.0\uid__1-312^DesignRootModel_PCB_ESP32-C3-MINI-1_V1(2)_PCB_ESP32.ipt
- C:\Users\micyg\Projects\virtual_pet\VirtualBlob\Mechanical\boards\MainBoard\MainBoard_0_4_0\VirtualBlob_MainBoard_0.4.0\VirtualBlob_MainBoard_0.4.0\uid__1-313^DesignRootModel_PCB_ESP32-C3-MINI-1_V1(2)_PCB_ESP32.ipt
- C:\Users\micyg\Projects\virtual_pet\VirtualBlob\Mechanical\boards\MainBoard\MainBoard_0_4_0\VirtualBlob_MainBoard_0.4.0\VirtualBlob_MainBoard_0.4.0\uid__1-314^DesignRootModel_PCB_ESP32-C3-MINI-1_V1(2)_PCB_ESP32.ipt
- C:\Users\micyg\Projects\virtual_pet\VirtualBlob\Mechanical\boards\MainBoard\MainBoard_0_4_0\VirtualBlob_MainBoard_0.4.0\VirtualBlob_MainBoard_0.4.0\uid__1-315^DesignRootModel_PCB_ESP32-C3-MINI-1_V1(2)_PCB_ESP32.ipt
- C:\Users\micyg\Projects\virtual_pet\VirtualBlob\Mechanical\boards\MainBoard\MainBoard_0_4_0\VirtualBlob_MainBoard_0.4.0\VirtualBlob_MainBoard_0.4.0\uid__1-316^DesignRootModel_PCB_ESP32-C3-MINI-1_V1(2)_PCB_ESP32.ipt
- C:\Users\micyg\Projects\virtual_pet\VirtualBlob\Mechanical\boards\MainBoard\MainBoard_0_4_0\VirtualBlob_MainBoard_0.4.0\VirtualBlob_MainBoard_0.4.0\uid__1-317^DesignRootModel_PCB_ESP32-C3-MINI-1_V1(2)_PCB_ESP32.ipt
- C:\Users\micyg\Projects\virtual_pet\VirtualBlob\Mechanical\boards\MainBoard\MainBoard_0_4_0\VirtualBlob_MainBoard_0.4.0\VirtualBlob_MainBoard_0.4.0\uid__1-318^DesignRootModel_PCB_ESP32-C3-MINI-1_V1(2)_PCB_ESP32.ipt
- C:\Users\micyg\Projects\virtual_pet\VirtualBlob\Mechanical\boards\MainBoard\MainBoard_0_4_0\VirtualBlob_MainBoard_0.4.0\VirtualBlob_MainBoard_0.4.0\uid__1-319^DesignRootModel_PCB_ESP32-C3-MINI-1_V1(2)_PCB_ESP32.ipt
- C:\Users\micyg\Projects\virtual_pet\VirtualBlob\Mechanical\boards\MainBoard\MainBoard_0_4_0\VirtualBlob_MainBoard_0.4.0\VirtualBlob_MainBoard_0.4.0\uid__1-320^DesignRootModel_PCB_ESP32-C3-MINI-1_V1(2)_PCB_ESP32.ipt
- C:\Users\micyg\Projects\virtual_pet\VirtualBlob\Mechanical\boards\MainBoard\MainBoard_0_4_0\VirtualBlob_MainBoard_0.4.0\VirtualBlob_MainBoard_0.4.0\uid__1-321^DesignRootModel_PCB_ESP32-C3-MINI-1_V1(2)_PCB_ESP32.ipt
- C:\Users\micyg\Projects\virtual_pet\VirtualBlob\Mechanical\boards\MainBoard\MainBoard_0_4_0\VirtualBlob_MainBoard_0.4.0\VirtualBlob_MainBoard_0.4.0\uid__1-322^DesignRootModel_PCB_ESP32-C3-MINI-1_V1(2)_PCB_ESP32.ipt
- C:\Users\micyg\Projects\virtual_pet\VirtualBlob\Mechanical\boards\MainBoard\MainBoard_0_4_0\VirtualBlob_MainBoard_0.4.0\VirtualBlob_MainBoard_0.4.0\uid__1-323^DesignRootModel_PCB_ESP32-C3-MINI-1_V1(2)_PCB_ESP32.ipt
- C:\Users\micyg\Projects\virtual_pet\VirtualBlob\Mechanical\boards\MainBoard\MainBoard_0_4_0\VirtualBlob_MainBoard_0.4.0\VirtualBlob_MainBoard_0.4.0\uid__1-324^DesignRootModel_PCB_ESP32-C3-MINI-1_V1(2)_PCB_ESP32.ipt
- C:\Users\micyg\Projects\virtual_pet\VirtualBlob\Mechanical\boards\MainBoard\MainBoard_0_4_0\VirtualBlob_MainBoard_0.4.0\VirtualBlob_MainBoard_0.4.0\uid__1-325^DesignRootModel_PCB_ESP32-C3-MINI-1_V1(2)_PCB_ESP32.ipt
- C:\Users\micyg\Projects\virtual_pet\VirtualBlob\Mechanical\boards\MainBoard\MainBoard_0_4_0\VirtualBlob_MainBoard_0.4.0\VirtualBlob_MainBoard_0.4.0\uid__1-326^DesignRootModel_PCB_ESP32-C3-MINI-1_V1(2)_PCB_ESP32.ipt
- C:\Users\micyg\Projects\virtual_pet\VirtualBlob\Mechanical\boards\MainBoard\MainBoard_0_4_0\VirtualBlob_MainBoard_0.4.0\VirtualBlob_MainBoard_0.4.0\uid__1-327^DesignRootModel_PCB_ESP32-C3-MINI-1_V1(2)_PCB_ESP32.ipt
- C:\Users\micyg\Projects\virtual_pet\VirtualBlob\Mechanical\boards\MainBoard\MainBoard_0_4_0\VirtualBlob_MainBoard_0.4.0\VirtualBlob_MainBoard_0.4.0\uid__1-328^DesignRootModel_PCB_ESP32-C3-MINI-1_V1(2)_PCB_ESP32.ipt
- C:\Users\micyg\Projects\virtual_pet\VirtualBlob\Mechanical\boards\MainBoard\MainBoard_0_4_0\VirtualBlob_MainBoard_0.4.0\VirtualBlob_MainBoard_0.4.0\uid__1-329^DesignRootModel_PCB_ESP32-C3-MINI-1_V1(2)_PCB_ESP32.ipt
- C:\Users\micyg\Projects\virtual_pet\VirtualBlob\Mechanical\boards\MainBoard\MainBoard_0_4_0\VirtualBlob_MainBoard_0.4.0\VirtualBlob_MainBoard_0.4.0\uid__2428^DesignRootModel_PCB_ESP32-C3-MINI-1_V1(2)_PCB_ESP32-.ipt
## Components (332 placed, 332 different names)
1. 33 [sub-assembly]
2. 36 [sub-assembly]
3. 47 [sub-assembly]
4. 50 [sub-assembly]
5. 53 [sub-assembly]
6. 56 [sub-assembly]
7. 59 [sub-assembly]
8. 62 [sub-assembly]
9. 65 [sub-assembly]
10. 68 [sub-assembly]
11. 71 [sub-assembly]
12. 74 [sub-assembly]
13. 77 [sub-assembly]
14. 80 [sub-assembly]
15. 83 [sub-assembly]
16. 86 [sub-assembly]
17. 89 [sub-assembly]
18. 92 [sub-assembly]
19. 95 [sub-assembly]
20. 98 [sub-assembly]
21. 101 [sub-assembly]
22. 102
23. 103
24. 104
25. 105
26. 106
27. 107
28. 108
29. 109
30. 110
31. 111
32. 112
33. 113
34. 114
35. 115
36. 116
37. 117
38. 118
39. 119
40. 120
41. 121
42. 122
43. 123
44. 124
45. 125
46. 126
47. 127
48. 128
49. 129
50. 130
51. 131
52. 132
53. 133
54. 134
55. 135
56. 136
57. 137
58. 138
59. 139
60. 140
61. 141
62. 142
63. 143
64. 144
65. 145
66. 146
67. 147
68. 148
69. 149
70. 150
71. 151
72. 152
73. 153
74. 154
75. 155
76. 156
77. 157
78. 158
79. 159
80. 160
81. 161
82. 162
83. 163
84. 164
85. 165
86. 166
87. 167
88. 168
89. 169
90. 170
91. 171
92. 172
93. 173
94. 174
95. 175
96. 176
97. 177
98. 178
99. 179
100. 180
101. 181
102. 182
103. 183
104. 184
105. 185
106. 186
107. 187
108. 188
109. 189
110. 190
111. 191
112. 192
113. 193
114. 194
115. 195
116. 196
117. 197
118. 198
119. 199
120. 200
121. 201
122. 202
123. 203
124. 204
125. 205
126. 206
127. 207
128. 208
129. 209
130. 210
131. 211
132. 212
133. 213
134. 214
135. 215
136. 216
137. 217
138. 218
139. 219
140. 220
141. 221
142. 222
143. 223
144. 224
145. 225
146. 226
147. 227
148. 228
149. 229
150. 230
151. 231
152. 232
153. 233
154. 234
155. 235
156. 236
157. 237
158. 238
159. 239
160. 240
161. 241
162. 242
163. 243
164. 244
165. 245
166. 246
167. 247
168. 248
169. 249
170. 250
171. 251
172. 252
173. 253
174. 254
175. 255
176. 256
177. 257
178. 258
179. 259
180. 260
181. 261
182. 262
183. 263
184. 264
185. 265
186. 266
187. 267
188. 268
189. 269
190. 270
191. 271
192. 272
193. 273
194. 274
195. 275
196. 276
197. 277
198. 278
199. 279
200. 280
201. 281
202. 282
203. 283
204. 284
205. 285
206. 286
207. 287
208. 288
209. 289
210. 290
211. 291
212. 292
213. 293
214. 294
215. 295
216. 296
217. 297
218. 298
219. 299
220. 300
221. 301
222. 302
223. 303
224. 304
225. 305
226. 306
227. 307
228. 308
229. 309
230. 310
231. 311
232. 312
233. 313
234. 314
235. 315
236. 316
237. 317
238. 318
239. 319
240. 320
241. 321
242. 322
243. 323
244. 324
245. 325
246. 326
247. 327
248. 328
249. 329
250. 330
251. 331
252. 332
253. 333
254. 334
255. 335
256. 336
257. 337
258. 338
259. 339
260. 340
261. 341
262. 342
263. 343
264. 344
265. 345
266. 346
267. 347
268. 348
269. 349
270. 350
271. 351
272. 352
273. 353
274. 354